# Autodesk Inventor assembly: Assembly3
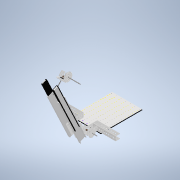
[picture p0: Inventor's stored thumbnail of the model, 180x180]
Saved by Autodesk Inventor 2020 (Build 240168000, 168)
## iProperties
Created: 2019-09-25
Part Number: Assembly3
Document SubType Name: Assembly
Designer: tbloo
Author: tbloo
## Documents named in this file (14)
- D:\Documents\GitHub\AO_Robotics\CAD\Projects\Timothy Bloot\Assembly3.iam
- D:\Documents\GitHub\AO_Robotics\CAD\Parts Kits\FTC Tetrix KOP Organized (7-24-19)\Frame Hardware\Tetrix_39066.ipt
- D:\Documents\GitHub\AO_Robotics\CAD\Parts Kits\FTC Tetrix KOP Organized (7-24-19)\Frame Hardware\Tetrix_39065.ipt
- D:\Documents\GitHub\AO_Robotics\CAD\Projects\Timothy Bloot\14in-slide-pt_1.ipt
- D:\Documents\GitHub\AO_Robotics\CAD\Projects\Timothy Bloot\14in-slide-pt_2.ipt
- D:\Documents\GitHub\AO_Robotics\CAD\Projects\Timothy Bloot\14in-slide-pt_3.ipt
- D:\Documents\GitHub\AO_Robotics\CAD\Parts Kits\Created Models\Base Plate.ipt
- D:\Documents\GitHub\AO_Robotics\CAD\Parts Kits\FTC Tetrix KOP Organized (7-24-19)\Frame Hardware\Tetrix_39067.ipt
- D:\Documents\GitHub\AO_Robotics\CAD\Parts Kits\FTC Tetrix KOP Organized (7-24-19)\Axle Hardware\Tetrix_39091.ipt
- D:\Documents\GitHub\AO_Robotics\CAD\Parts Kits\FTC Tetrix KOP Organized (7-24-19)\Axle Hardware\Tetrix_39088.ipt
- D:\Documents\GitHub\AO_Robotics\CAD\Parts Kits\FTC Tetrix KOP Organized (7-24-19)\Axle Hardware\Tetrix_39172.iam
- D:\Documents\GitHub\AO_Robotics\CAD\Parts Kits\FTC Tetrix KOP Organized (7-24-19)\Gear\Tetrix_39169.ipt
- D:\Documents\GitHub\AO_Robotics\CAD\Parts Kits\FTC Tetrix KOP Organized (7-24-19)\Gear\Tetrix_38007_Gear.ipt
- D:\Documents\GitHub\AO_Robotics\CAD\Parts Kits\FTC Tetrix KOP Organized (7-24-19)\Gear\Tetrix_38007_Bearing.ipt
## Components (34 placed, 13 different names)
1. Tetrix_39066:1 — Rigid:1, Rigid:3, Mate:1, Flush:3, Flush:4
2. Tetrix_39066:2 — Rigid:2, Rigid:3, Mate:2, Flush:1, Flush:2
3. Tetrix_39065:1 — Rigid:1, Rigid:10
4. Tetrix_39065:2 — Rigid:2, Rigid:11
5. 14in-slide-pt_1:1 — Mate:1, Flush:3, Flush:4
6. 14in-slide-pt_2:1
7. 14in-slide-pt_3:1
8. 14in-slide-pt_1:2 — Mate:2, Flush:1, Flush:2, Mate:3
9. 14in-slide-pt_2:2
10. 14in-slide-pt_3:2
11. Base Plate:1
12. Tetrix_39067:1
13. Tetrix_39067:2
14. Tetrix_39066:3
15. Tetrix_39066:4
16. Tetrix_39091:1
17. Tetrix_39091:2 — Mate:3
18. Tetrix_39091:3 — Cylindrical:1
19. Tetrix_39091:4
20. Tetrix_39088:1 — Rigid:12
21. Tetrix_39172:1 [sub-assembly]
22. Tetrix_39169:1
23. Tetrix_39172:2 [sub-assembly] — Rigid:10, Rigid:13
24. Tetrix_39172:3 [sub-assembly] — Rigid:11, Rigid:12
25. Tetrix_39088:2 — Rigid:13, Cylindrical:1
26. Tetrix_38007_Gear:1 — Rotational:9
27. Tetrix_38007_Gear:2 — Rotational:10
28. Tetrix_38007_Bearing:1 — Rotational:10, Rotational:14
29. Tetrix_38007_Bearing:2 — Rotational:9, Rotational:13
30. Tetrix_39065:3 — Rotational:5, Rotational:6, Rotational:11, Rotational:12
31. Tetrix_39088:3 — Rotational:5
32. Tetrix_39088:4 — Rotational:6
33. Tetrix_39091:5 — Rotational:11, Rotational:14
34. Tetrix_39091:6 — Rotational:12, Rotational:13
## Relationships (39: WeldJoint 12, RevoluteJoint 12, Flush 7, TranslationJoint 4, Mate 3, CylindricalJoint 1)
- Rigid:1 [WeldJoint]: Tetrix_39066:1 ↔ Tetrix_39065:1
- Rigid:2 [WeldJoint]: Tetrix_39066:2 ↔ Tetrix_39065:2
- Rigid:3 [WeldJoint]: Tetrix_39066:1 ↔ Tetrix_39066:2
- [TranslationJoint]: 14in-slide-pt_1:1 ↔ 14in-slide-pt_2:1
- [TranslationJoint]: 14in-slide-pt_2:1 ↔ 14in-slide-pt_3:1
- [TranslationJoint]: 14in-slide-pt_1:2 ↔ 14in-slide-pt_2:2
- [TranslationJoint]: 14in-slide-pt_2:2 ↔ 14in-slide-pt_3:2
- Mate:1: Tetrix_39066:1 ↔ 14in-slide-pt_1:1
- Mate:2: Tetrix_39066:2 ↔ 14in-slide-pt_1:2
- Flush:1: Tetrix_39066:2 ↔ 14in-slide-pt_1:2
- Flush:2: Tetrix_39066:2 ↔ 14in-slide-pt_1:2
- Flush:3: Tetrix_39066:1 ↔ 14in-slide-pt_1:1
- Flush:4: Tetrix_39066:1 ↔ 14in-slide-pt_1:1
- [WeldJoint]: Base Plate:1 ↔ Tetrix_39067:1
- [WeldJoint]: Base Plate:1 ↔ Tetrix_39067:2
- [WeldJoint]: Base Plate:1 ↔ Tetrix_39066:4
- [Flush]: Tetrix_39067:1 ↔ Tetrix_39066:3
- [Flush]: Tetrix_39067:1 ↔ Tetrix_39066:3
- [Flush]: Tetrix_39067:1 ↔ Tetrix_39066:3
- [RevoluteJoint]: Tetrix_39066:3 ↔ Tetrix_39091:1
- [WeldJoint]: Tetrix_39066:4 ↔ Tetrix_39091:2
- [RevoluteJoint]: Tetrix_39066:3 ↔ Tetrix_39091:3
- [RevoluteJoint]: Tetrix_39066:4 ↔ Tetrix_39091:4
- [WeldJoint]: Tetrix_39172:1 ↔ Tetrix_39169:1
- [RevoluteJoint] (1.4 mm): Tetrix_39066:4 ↔ Tetrix_39172:1
- Rigid:10 [WeldJoint]: Tetrix_39065:1 ↔ Tetrix_39172:2
- Rigid:11 [WeldJoint]: Tetrix_39065:2 ↔ Tetrix_39172:3
- Rigid:12 [WeldJoint]: Tetrix_39088:1 ↔ Tetrix_39172:3
- Rigid:13 [WeldJoint]: Tetrix_39172:2 ↔ Tetrix_39088:2
- Cylindrical:1: Tetrix_39091:3 ↔ Tetrix_39088:2
- Mate:3: 14in-slide-pt_1:2 ↔ Tetrix_39091:2
- Rotational:5 [RevoluteJoint]: Tetrix_39065:3 ↔ Tetrix_39088:3
- Rotational:6 [RevoluteJoint]: Tetrix_39065:3 ↔ Tetrix_39088:4
- Rotational:9 [RevoluteJoint]: Tetrix_38007_Gear:1 ↔ Tetrix_38007_Bearing:2
- Rotational:10 [RevoluteJoint]: Tetrix_38007_Gear:2 ↔ Tetrix_38007_Bearing:1
- Rotational:11 [RevoluteJoint]: Tetrix_39065:3 ↔ Tetrix_39091:5
- Rotational:12 [RevoluteJoint]: Tetrix_39065:3 ↔ Tetrix_39091:6
- Rotational:13 [RevoluteJoint]: Tetrix_38007_Bearing:2 ↔ Tetrix_39091:6
- Rotational:14 [RevoluteJoint]: Tetrix_38007_Bearing:1 ↔ Tetrix_39091:5
## Named parameters: d3_d2 = 0 mm, d11_d2 = 0 mm, d12_d3 = 0 mm, d13_d4 = -99.7691 mm, d14_d5 = -177.8 mm, d15_d6 = 0 mm, d16_d7 = 0 mm, d17_d8 = 0 mm, d18_d9 = -177.8 mm
